# Autodesk Inventor assembly: driven wheel assembly
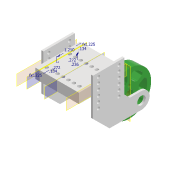
[picture p0: Inventor's stored thumbnail of the model, 180x180]
Saved by Autodesk Inventor 2020 (Build 240168000, 168)
## iProperties
Created: 2020-01-25
Part Number: driven wheel assembly
Document SubType Name: Assembly
Designer: ball
Author: ball
## Documents named in this file (4)
- C:\FTC\FTC8863CAD\2019 Robot\Collection\Intake\driven wheel assembly.iam
- C:\FTC\FTC8863CAD\2019 Robot\general robot componets\pulley .25 in + wheel.2.iam
- C:\FTC\FTC8863CAD\2019 Robot\Collection\Intake\driven wheel arm angled adjustable holes.ipt
- C:\FTC\FTC8863CAD\2019 Robot\Collection\Intake\driven wheel mount to xrail adjustable holes.ipt
## Components (4 placed, 3 different names)
1. driven wheel mount to xrail adjustable holes:1 — Mate:1, Mate:2, Mate:3, Mate:4
2. pulley .25 in + wheel.2:1 [sub-assembly] — Mate:5, Mate:6
3. driven wheel arm angled adjustable holes:1 — Mate:1, Mate:2, Mate:3, Flush:1, Mate:6
4. driven wheel arm angled adjustable holes:2 — Mate:4, Flush:1, Mate:5
## Relationships (7: Mate 6, Flush 1)
- Mate:1: driven wheel mount to xrail adjustable holes:1 ↔ driven wheel arm angled adjustable holes:1
- Mate:2: driven wheel mount to xrail adjustable holes:1 ↔ driven wheel arm angled adjustable holes:1
- Mate:3: driven wheel mount to xrail adjustable holes:1 ↔ driven wheel arm angled adjustable holes:1
- Mate:4: driven wheel mount to xrail adjustable holes:1 ↔ driven wheel arm angled adjustable holes:2
- Flush:1: driven wheel arm angled adjustable holes:1 ↔ driven wheel arm angled adjustable holes:2
- Mate:5 (12.7 mm): pulley .25 in + wheel.2:1 ↔ driven wheel arm angled adjustable holes:2
- Mate:6: pulley .25 in + wheel.2:1 ↔ driven wheel arm angled adjustable holes:1
